# Autodesk Inventor assembly: Assembly1
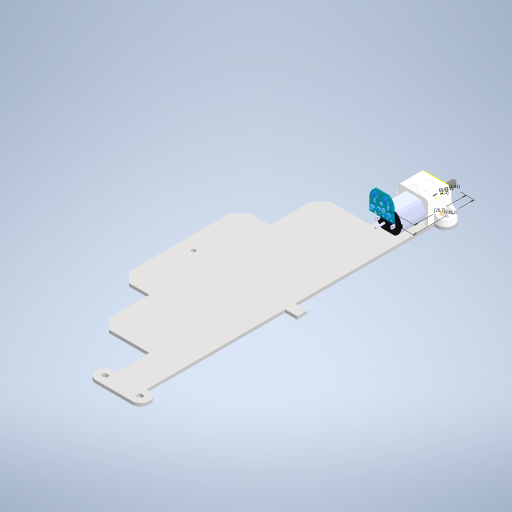
[picture p0: Inventor's stored thumbnail of the model, 512x512]
Saved by Autodesk Inventor 2024 (Build 280153000, 153)
## iProperties
Created: 2024-09-23
Part Number: Assembly1
Document SubType Name: Assembly
Designer: kamil
Author: kamil
## Documents named in this file (4)
- D:\Projects\Robotics\MaxVoltstapenV2\PCB\2ndVersion\Assembly1.iam
- D:\Projects\Robotics\MaxVoltstapenV2\3DModel\linefollower_chassy_model.ipt
- D:\Projects\Robotics\MaxVoltstapenV2\3DModel\parts\micro-metal-gearmotor-extended-with-1086-bracket\micro-metal-gearmotor-extended-with-1086-bracket.ipt
- D:\Projects\Robotics\MaxVoltstapenV2\3DModel\parts\magnetic-encoder-pair-kit-for-micro-metal-gearmotors-hpcb-compatible-enc03b\magnetic-encoder-pair-kit-for-micro-metal-gearmotors-hpcb-compatible-enc03b.ipt
## Components (3 placed, 3 different names)
1. linefollower_chassy_model:1 — Mate:1, Mate:2, Mate:3
2. micro-metal-gearmotor-extended-with-1086-bracket:1 — Mate:1, Mate:2, Mate:3
3. magnetic-encoder-pair-kit-for-micro-metal-gearmotors-hpcb-compatible-enc03b:1
## Relationships (3: Mate 3)
- Mate:1: linefollower_chassy_model:1 ↔ micro-metal-gearmotor-extended-with-1086-bracket:1
- Mate:2: linefollower_chassy_model:1 ↔ micro-metal-gearmotor-extended-with-1086-bracket:1
- Mate:3: linefollower_chassy_model:1 ↔ micro-metal-gearmotor-extended-with-1086-bracket:1
